# Autodesk Inventor assembly: linkage_system_test_3
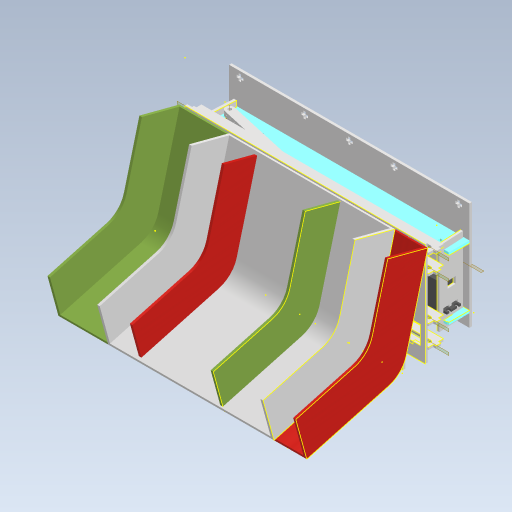
[picture p0: Inventor's stored thumbnail of the model, 512x512]
Saved by Autodesk Inventor 2023 (Build 270158000, 158)
## iProperties
Created: 2023-06-08
Part Number: linkage_system_test_3
Document SubType Name: Assembly
Designer: JOU
Author: JOU
## Documents named in this file (16)
- C:\Users\JOU\Desktop\git\Areo_Rider_Cabin\Expansion\test\linkage_system_test_3.iam
- C:\Users\JOU\Desktop\git\Areo_Rider_Cabin\Expansion\test\plate_expansion.ipt
- C:\Users\JOU\Desktop\git\Areo_Rider_Cabin\Expansion\test\零件1.ipt
- C:\Users\JOU\Desktop\git\Areo_Rider_Cabin\Expansion\test\零件8.ipt
- C:\Users\JOU\Desktop\git\Areo_Rider_Cabin\Expansion\test\零件4.ipt
- C:\Users\JOU\Desktop\git\Areo_Rider_Cabin\Expansion\test\零件5.ipt
- C:\Users\JOU\Desktop\git\Areo_Rider_Cabin\Expansion\test\零件7.ipt
- C:\Users\JOU\Desktop\git\Areo_Rider_Cabin\car\外抓檔\Tower Pro MG996R.ipt
- C:\Users\JOU\Desktop\git\Areo_Rider_Cabin\Expansion\test\adjustable_130.ipt
- C:\Users\JOU\Desktop\git\Areo_Rider_Cabin\Expansion\test\adjustable_200.ipt
- C:\Users\JOU\Desktop\git\Areo_Rider_Cabin\Expansion\test\零件12.ipt
- C:\Users\JOU\Desktop\git\Areo_Rider_Cabin\Expansion\test\adjustable_80.ipt
- C:\Users\JOU\Desktop\git\Areo_Rider_Cabin\Expansion\test\零件13.ipt
- C:\Users\JOU\Desktop\git\Areo_Rider_Cabin\Airfoil & Nuzzle\sus_1.ipt
- C:\Users\JOU\Desktop\git\Areo_Rider_Cabin\Airfoil & Nuzzle\sus_2.ipt
- C:\Users\JOU\Desktop\git\Areo_Rider_Cabin\Airfoil & Nuzzle\splitter.ipt
## Components (34 placed, 15 different names)
1. plate_expansion:1
2. 零件1:1
3. 零件8:1
4. 零件4:1
5. 零件4:2
6. 零件4:3
7. 零件4:4
8. 零件5:1
9. 零件7:1
10. 零件7:2 — 貼合:44
11. 零件8:2
12. Tower Pro MG996R:1
13. Tower Pro MG996R:2
14. 零件1:2 — 插入:20
15. adjustable_130:1
16. adjustable_200:1 — 插入:21
17. adjustable_200:2
18. adjustable_200:3
19. adjustable_200:4
20. adjustable_200:5
21. adjustable_200:6
22. adjustable_200:7
23. adjustable_200:8
24. 零件12:1
25. adjustable_80:1
26. adjustable_130:2
27. 零件12:2
28. adjustable_80:2
29. 零件13:1 — 插入:20, 插入:21
30. sus_1:1 — 貼合:42, 貼合:43, 齊平:11
31. sus_2:1 — 貼合:40, 貼合:41, 齊平:10, 貼合:44
32. splitter:1 — 貼合:37, 貼合:39, 貼合:42, 貼合:43, 齊平:11
33. splitter:2 — 貼合:36, 貼合:38
34. splitter:3 — 貼合:36, 貼合:37, 貼合:38, 貼合:39, 貼合:40, 貼合:41, 齊平:10
## Relationships (77: Mate 44, Insert 21, Flush 11, Angle 1)
- [Mate]: plate_expansion:1 ↔ 零件1:1
- [Flush]: plate_expansion:1 ↔ 零件1:1
- [Mate]: plate_expansion:1 ↔ 零件1:1
- [Mate]: 零件1:1 ↔ 零件8:1
- [Mate]: 零件1:1 ↔ 零件8:1
- [Flush]: 零件4:2 ↔ 零件4:4
- [Flush]: 零件4:1 ↔ 零件4:2
- [Flush]: 零件4:1 ↔ 零件4:3
- [Flush]: 零件4:1 ↔ 零件5:1
- [Mate]: 零件4:1 ↔ 零件5:1
- [Mate]: 零件4:3 ↔ 零件5:1
- [Mate]: 零件4:2 ↔ 零件5:1
- [Mate]: 零件4:4 ↔ 零件5:1
- [Mate]: 零件4:3 ↔ 零件5:1
- [Angle] (0 deg): plate_expansion:1 ↔ 零件5:1
- [Flush]: plate_expansion:1 ↔ 零件5:1
- [Mate]: 零件5:1 ↔ 零件7:1
- [Mate]: 零件5:1 ↔ 零件7:1
- [Mate]: 零件5:1 ↔ 零件7:1
- [Mate]: 零件5:1 ↔ 零件7:2
- [Mate]: 零件5:1 ↔ 零件7:2
- [Mate]: 零件5:1 ↔ 零件7:2
- [Mate]: 零件1:1 ↔ 零件8:2
- [Insert]: 零件1:1 ↔ Tower Pro MG996R:2
- [Mate]: plate_expansion:1 ↔ 零件1:2
- [Flush]: plate_expansion:1 ↔ 零件1:2
- [Flush]: 零件1:1 ↔ 零件1:2
- [Insert]: Tower Pro MG996R:1 ↔ 零件1:2
- [Mate]: 零件8:1 ↔ Tower Pro MG996R:1
- [Mate]: 零件8:2 ↔ Tower Pro MG996R:2
- [Mate]: 零件1:1 ↔ 零件8:2
- [Mate]: 零件4:1 ↔ 零件5:1
- [Mate]: 零件4:2 ↔ 零件5:1
- [Mate]: 零件4:4 ↔ 零件5:1
- [Insert]: adjustable_200:1 ↔ adjustable_200:2
- [Insert]: adjustable_200:1 ↔ adjustable_200:2
- [Mate]: 零件1:2 ↔ adjustable_200:1
- [Insert]: adjustable_200:3 ↔ adjustable_200:4
- [Insert]: adjustable_200:3 ↔ adjustable_200:4
- [Insert]: adjustable_200:5 ↔ adjustable_200:6
- [Insert]: adjustable_200:5 ↔ adjustable_200:6
- [Insert]: adjustable_200:7 ↔ adjustable_200:8
- [Insert]: adjustable_200:7 ↔ adjustable_200:8
- [Mate]: Tower Pro MG996R:2 ↔ adjustable_200:4
- [Mate] (3.87 mm): 零件1:1 ↔ adjustable_200:3
- [Insert]: 零件1:1 ↔ adjustable_200:7
- [Mate]: Tower Pro MG996R:1 ↔ adjustable_200:6
- [Mate] (3.87 mm): 零件1:2 ↔ adjustable_200:6
- [Mate]: 零件4:3 ↔ 零件12:1
- [Insert]: adjustable_80:1 ↔ 零件12:2
- [Insert]: adjustable_80:1 ↔ adjustable_130:2
- [Insert]: adjustable_200:6 ↔ 零件12:2
- [Insert]: adjustable_200:6 ↔ adjustable_130:2
- [Insert]: adjustable_200:1 ↔ 零件12:1
- [Insert]: adjustable_130:1 ↔ adjustable_200:1
- [Insert]: adjustable_130:1 ↔ adjustable_80:2
- [Insert]: 零件12:1 ↔ adjustable_80:2
- [Mate]: 零件4:3 ↔ 零件12:1
- [Mate]: 零件4:3 ↔ 零件12:2
- [Mate]: 零件4:3 ↔ 零件12:2
- [Mate]: 零件4:4 ↔ adjustable_200:4
- [Mate]: 零件4:2 ↔ adjustable_200:7
- [Flush]: adjustable_130:1 ↔ adjustable_130:2
- [Mate]: 零件4:3 ↔ adjustable_200:5
- 插入:20 [Insert]: 零件1:2 ↔ 零件13:1
- 插入:21 [Insert]: adjustable_200:1 ↔ 零件13:1
- 貼合:36 [Mate]: splitter:2 ↔ splitter:3
- 貼合:37 [Mate]: splitter:1 ↔ splitter:3
- 貼合:38 [Mate]: splitter:2 ↔ splitter:3
- 貼合:39 [Mate]: splitter:1 ↔ splitter:3
- 貼合:40 [Mate]: sus_2:1 ↔ splitter:3
- 貼合:41 [Mate]: sus_2:1 ↔ splitter:3
- 貼合:42 [Mate]: sus_1:1 ↔ splitter:1
- 貼合:43 [Mate]: sus_1:1 ↔ splitter:1
- 齊平:10 [Flush] (20 mm): sus_2:1 ↔ splitter:3
- 齊平:11 [Flush] (20 mm): sus_1:1 ↔ splitter:1
- 貼合:44 [Mate]: 零件7:2 ↔ sus_2:1
## Named parameters: d455_d451 = 0 mm, d456_d452 = 0 mm, d437_d433 = 0 mm, d438_d434 = 0 mm, d439_d437_d433 = 0 mm, d440_d438_d434 = 0 mm, d441_d437_d433 = 0 mm, d442_d438_d434 = 0 mm
